# Autodesk Inventor assembly: SimpleBase_v1
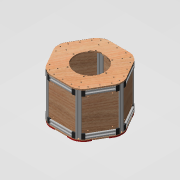
[picture p0: Inventor's stored thumbnail of the model, 180x180]
Saved by Autodesk Inventor 2016 (Build 200138000, 138)
## iProperties
Created: 2015-02-21
Part Number: SimpleBase_v1
Document SubType Name: Assembly
Designer: 4ndreas
Author: 4ndreas
## Documents named in this file (11)
- C:\Users\4ndreas\Documents\Inventor\RobotARM v2\v3\SimpleBase_v1.iam
- C:\Users\4ndreas\Documents\Inventor\RobotARM v2\Base\SimpleBase_Segment.iam
- C:\Users\4ndreas\Documents\Inventor\RobotARM v2\Base\BottomBase_Full.ipt
- C:\Users\4ndreas\Documents\Inventor\RobotARM v2\Base\TopBase_Full.ipt
- C:\Users\4ndreas\Documents\Inventor\RobotARM v2\Base\Mount_Pi2_B+.ipt
- C:\Users\4ndreas\Documents\Inventor\RobotARM v2\Base\Moterboard_Mount.ipt
- C:\Users\4ndreas\Documents\Inventor\RobotARM v2\Base\MotorDriverMount.ipt
- C:\Users\4ndreas\Documents\Inventor\RobotARM v2\Base\BaseTop.ipt
- C:\Users\4ndreas\Documents\Inventor\RobotARM v2\Base\BaseFeet.ipt
- C:\Users\4ndreas\Documents\Inventor\Content Center Files\R2014\de-DE\DIN 7991(2)\DIN 7991 - M4x8.ipt
- C:\Users\4ndreas\Documents\Inventor\Content Center Files\R2014\de-DE\DIN 7991(2)\DIN 7991 - M6x30.ipt
## Components (43 placed, 10 different names)
1. SimpleBase_Segment:1 [sub-assembly] — Passend:1, Passend:2, Fluchtend:1, Fluchtend:5, Passend:3, Passend:4, Passend:29, Passend:35, Passend:36, Passend:46
2. SimpleBase_Segment:2 [sub-assembly] — Passend:1, Passend:2, Fluchtend:1, Fluchtend:2, Fluchtend:3, Passend:13, Passend:17, Passend:21, Passend:22
3. SimpleBase_Segment:3 [sub-assembly] — Fluchtend:2, Passend:9, Passend:10, Passend:12, Passend:14
4. SimpleBase_Segment:4 [sub-assembly] — Fluchtend:3, Fluchtend:4, Passend:7, Passend:8, Passend:9, Passend:10, Passend:15
5. SimpleBase_Segment:5 [sub-assembly] — Fluchtend:4, Passend:5, Passend:6, Passend:7, Passend:8, Passend:11, Passend:18, Passend:23, Passend:30, Passend:31, Passend:32
6. SimpleBase_Segment:6 [sub-assembly] — Fluchtend:5, Passend:3, Passend:4, Passend:5, Passend:6, Passend:28, Passend:33, Passend:34
7. BottomBase_Full:1 — Passend:21, Passend:22, Passend:23, Passend:37, Passend:38, Passend:39, Passend:41, Passend:42, Passend:43, Passend:44, Passend:45
8. TopBase_Full:1 — Passend:15, Passend:16, Passend:17, Passend:18, Passend:19, Passend:20
9. TopBase_Full:2 — Passend:16, Passend:19, Passend:20
10. Mount_Pi2_B+:1 — Passend:28, Passend:33, Passend:34
11. Moterboard_Mount:1 — Passend:29, Passend:35, Passend:36
12. MotorDriverMount:1 — Passend:30, Passend:31, Passend:32
13. BaseTop:1 — Passend:37, Passend:38, Passend:39
14. BaseFeet:1 — Passend:41, Passend:42, Fluchtend:6, Fluchtend:7, Fluchtend:8, Fluchtend:9
15. DIN 7991 M4x8:3 — Passend:43, Fluchtend:6
16. DIN 7991 M4x8:1 — Passend:44, Fluchtend:7
17. DIN 7991 M6x30:1 — Passend:46, Fluchtend:9
18. DIN 7991 M4x8:2 — Passend:45, Fluchtend:8
19. BaseFeet:2
20. DIN 7991 M4x8:4
21. DIN 7991 M4x8:5
22. DIN 7991 M6x30:2
23. DIN 7991 M4x8:6
24. BaseFeet:3
25. DIN 7991 M4x8:7
26. DIN 7991 M4x8:8
27. DIN 7991 M6x30:3
28. DIN 7991 M4x8:9
29. BaseFeet:4
30. DIN 7991 M4x8:10
31. DIN 7991 M4x8:11
32. DIN 7991 M6x30:4
33. DIN 7991 M4x8:12
34. BaseFeet:5
35. DIN 7991 M4x8:13
36. DIN 7991 M4x8:14
37. DIN 7991 M6x30:5
38. DIN 7991 M4x8:15
39. BaseFeet:6
40. DIN 7991 M4x8:16
41. DIN 7991 M4x8:17
42. DIN 7991 M6x30:6
43. DIN 7991 M4x8:18
## Component patterns: (6 elements, first: BaseFeet:1 + DIN 7991 M4x8:3 + DIN 7991 M4x8:1 + DIN 7991 M6x30:1 + DIN 7991 M4x8:2)
## Relationships (50: Mate 41, Flush 9)
- Passend:1 [Mate]: SimpleBase_Segment:1 ↔ SimpleBase_Segment:2
- Passend:2 [Mate]: SimpleBase_Segment:1 ↔ SimpleBase_Segment:2
- Fluchtend:1 [Flush]: SimpleBase_Segment:1 ↔ SimpleBase_Segment:2
- Fluchtend:2 [Flush]: SimpleBase_Segment:2 ↔ SimpleBase_Segment:3
- Fluchtend:3 [Flush]: SimpleBase_Segment:2 ↔ SimpleBase_Segment:4
- Fluchtend:4 [Flush]: SimpleBase_Segment:4 ↔ SimpleBase_Segment:5
- Fluchtend:5 [Flush]: SimpleBase_Segment:1 ↔ SimpleBase_Segment:6
- Passend:3 [Mate]: SimpleBase_Segment:1 ↔ SimpleBase_Segment:6
- Passend:4 [Mate]: SimpleBase_Segment:1 ↔ SimpleBase_Segment:6
- Passend:5 [Mate]: SimpleBase_Segment:5 ↔ SimpleBase_Segment:6
- Passend:6 [Mate]: SimpleBase_Segment:5 ↔ SimpleBase_Segment:6
- Passend:7 [Mate]: SimpleBase_Segment:4 ↔ SimpleBase_Segment:5
- Passend:8 [Mate]: SimpleBase_Segment:4 ↔ SimpleBase_Segment:5
- Passend:9 [Mate]: SimpleBase_Segment:3 ↔ SimpleBase_Segment:4
- Passend:10 [Mate]: SimpleBase_Segment:3 ↔ SimpleBase_Segment:4
- Passend:11 [Mate] (3 mm): SimpleBase_Segment:5
- Passend:12 [Mate]: SimpleBase_Segment:3
- Passend:13 [Mate]: SimpleBase_Segment:2
- Passend:14 [Mate]: SimpleBase_Segment:3
- Passend:15 [Mate]: SimpleBase_Segment:4 ↔ TopBase_Full:1
- Passend:16 [Mate]: TopBase_Full:1 ↔ TopBase_Full:2
- Passend:17 [Mate]: SimpleBase_Segment:2 ↔ TopBase_Full:1
- Passend:18 [Mate]: SimpleBase_Segment:5 ↔ TopBase_Full:1
- Passend:19 [Mate]: TopBase_Full:1 ↔ TopBase_Full:2
- Passend:20 [Mate]: TopBase_Full:1 ↔ TopBase_Full:2
- Passend:21 [Mate]: SimpleBase_Segment:2 ↔ BottomBase_Full:1
- Passend:22 [Mate]: SimpleBase_Segment:2 ↔ BottomBase_Full:1
- Passend:23 [Mate]: SimpleBase_Segment:5 ↔ BottomBase_Full:1
- Passend:28 [Mate]: SimpleBase_Segment:6 ↔ Mount_Pi2_B+:1
- Passend:29 [Mate]: SimpleBase_Segment:1 ↔ Moterboard_Mount:1
- Passend:30 [Mate]: SimpleBase_Segment:5 ↔ MotorDriverMount:1
- Passend:31 [Mate]: SimpleBase_Segment:5 ↔ MotorDriverMount:1
- Passend:32 [Mate]: SimpleBase_Segment:5 ↔ MotorDriverMount:1
- Passend:33 [Mate]: SimpleBase_Segment:6 ↔ Mount_Pi2_B+:1
- Passend:34 [Mate]: SimpleBase_Segment:6 ↔ Mount_Pi2_B+:1
- Passend:35 [Mate]: SimpleBase_Segment:1 ↔ Moterboard_Mount:1
- Passend:36 [Mate]: SimpleBase_Segment:1 ↔ Moterboard_Mount:1
- Passend:37 [Mate]: BottomBase_Full:1 ↔ BaseTop:1
- Passend:38 [Mate]: BottomBase_Full:1 ↔ BaseTop:1
- Passend:39 [Mate]: BottomBase_Full:1 ↔ BaseTop:1
- Passend:41 [Mate]: BottomBase_Full:1 ↔ BaseFeet:1
- Passend:42 [Mate]: BottomBase_Full:1 ↔ BaseFeet:1
- Passend:43 [Mate]: BottomBase_Full:1 ↔ DIN 7991 M4x8:3
- Passend:44 [Mate]: BottomBase_Full:1 ↔ DIN 7991 M4x8:1
- Passend:45 [Mate]: BottomBase_Full:1 ↔ DIN 7991 M4x8:2
- Fluchtend:6 [Flush]: BaseFeet:1 ↔ DIN 7991 M4x8:3
- Fluchtend:7 [Flush]: BaseFeet:1 ↔ DIN 7991 M4x8:1
- Fluchtend:8 [Flush]: BaseFeet:1 ↔ DIN 7991 M4x8:2
- Passend:46 [Mate]: SimpleBase_Segment:1 ↔ DIN 7991 M6x30:1
- Fluchtend:9 [Flush]: BaseFeet:1 ↔ DIN 7991 M6x30:1
